# Autodesk Inventor assembly: HarmonicDrive
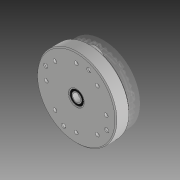
[picture p0: Inventor's stored thumbnail of the model, 180x180]
Saved by Autodesk Inventor 2020 (Build 240168000, 168)
## iProperties
Created: 2021-03-19
Part Number: HarmonicDrive
Document SubType Name: Assembly
Designer: DDeGo
Author: DDeGo
## Documents named in this file (10)
- C:\Users\DDeGo\Documents\Drew\Projects\OS-ARM\cad\HarmonicDrive75mm\HarmonicDrive.iam
- C:\Users\DDeGo\Documents\Drew\Projects\OS-ARM\cad\HarmonicDrive75mm\HD_housing.ipt
- C:\Users\DDeGo\Documents\Drew\Projects\OS-ARM\cad\HarmonicDrive75mm\HD_rotor.ipt
- C:\Users\DDeGo\Documents\Drew\Projects\OS-ARM\cad\OTS\608 bearing.ipt
- C:\Users\DDeGo\Documents\Drew\Projects\OS-ARM\cad\HarmonicDrive75mm\HD_housing2.ipt
- C:\Users\DDeGo\Documents\Drew\Projects\OS-ARM\cad\HarmonicDrive75mm\HD_Spacer.ipt
- C:\Users\DDeGo\Documents\Drew\Projects\OS-ARM\cad\HarmonicDrive75mm\HD_BearingShaft1.ipt
- C:\Users\DDeGo\Documents\Drew\Projects\OS-ARM\cad\HarmonicDrive75mm\HD_BearingShaft2.ipt
- C:\Users\DDeGo\Documents\Drew\Projects\OS-ARM\cad\HarmonicDrive75mm\HD_rotorshim.ipt
- C:\Users\DDeGo\Documents\Drew\Projects\OS-ARM\cad\OTS\688 bearing.ipt
## Components (18 placed, 9 different names)
1. HD_housing:1 — Mate:53, Mate:54, Mate:57, Mate:60
2. HD_rotor:1 — Mate:4, Mate:5, Mate:9, Mate:11, Mate:23, Mate:24, Rotation:1, Mate:45, Mate:46, Mate:49, Mate:50, Mate:61
3. HD_housing2:1 — Rotation:1, Mate:53, Mate:58, Mate:59, Mate:60
4. 608 bearing:2 — Mate:5, Mate:34, Mate:38, Mate:47
5. 608 bearing:3 — Mate:4, Mate:36, Mate:39, Mate:48
6. 608 bearing:5 — Mate:9, Mate:33, Mate:37, Mate:51
7. 608 bearing:6 — Mate:11, Mate:35, Mate:40, Mate:52
8. HD_Spacer:1 — Mate:23, Mate:24, Mate:62
9. HD_BearingShaft1:1 — Mate:35, Mate:40
10. HD_BearingShaft2:1 — Mate:33, Mate:37, Mate:41, Mate:42
11. HD_BearingShaft1:2 — Mate:36, Mate:39
12. HD_BearingShaft2:2 — Mate:34, Mate:38, Mate:43, Mate:44
13. HD_rotorshim:1 — Mate:41, Mate:49, Mate:51
14. HD_rotorshim:2 — Mate:42, Mate:50, Mate:52
15. HD_rotorshim:3 — Mate:43, Mate:45, Mate:47
16. HD_rotorshim:4 — Mate:44, Mate:46, Mate:48
17. 688 bearing:1 — Mate:54, Mate:57, Mate:61, Mate:62
18. 688 bearing:2 — Mate:58, Mate:59
## Relationships (35: Mate 34, RelateRotation 1)
- Mate:4: HD_rotor:1 ↔ 608 bearing:3
- Mate:5: HD_rotor:1 ↔ 608 bearing:2
- Mate:9: HD_rotor:1 ↔ 608 bearing:5
- Mate:11: HD_rotor:1 ↔ 608 bearing:6
- Mate:23: HD_rotor:1 ↔ HD_Spacer:1
- Mate:24: HD_rotor:1 ↔ HD_Spacer:1
- Rotation:1 [RelateRotation] (20.5 ul): HD_rotor:1 ↔ HD_housing2:1
- Mate:33: 608 bearing:5 ↔ HD_BearingShaft2:1
- Mate:34: 608 bearing:2 ↔ HD_BearingShaft2:2
- Mate:35: 608 bearing:6 ↔ HD_BearingShaft1:1
- Mate:36: 608 bearing:3 ↔ HD_BearingShaft1:2
- Mate:37: 608 bearing:5 ↔ HD_BearingShaft2:1
- Mate:38: 608 bearing:2 ↔ HD_BearingShaft2:2
- Mate:39: 608 bearing:3 ↔ HD_BearingShaft1:2
- Mate:40: 608 bearing:6 ↔ HD_BearingShaft1:1
- Mate:41: HD_BearingShaft2:1 ↔ HD_rotorshim:1
- Mate:42: HD_BearingShaft2:1 ↔ HD_rotorshim:2
- Mate:43: HD_BearingShaft2:2 ↔ HD_rotorshim:3
- Mate:44: HD_BearingShaft2:2 ↔ HD_rotorshim:4
- Mate:45: HD_rotor:1 ↔ HD_rotorshim:3
- Mate:46: HD_rotor:1 ↔ HD_rotorshim:4
- Mate:47: 608 bearing:2 ↔ HD_rotorshim:3
- Mate:48: 608 bearing:3 ↔ HD_rotorshim:4
- Mate:49: HD_rotor:1 ↔ HD_rotorshim:1
- Mate:50: HD_rotor:1 ↔ HD_rotorshim:2
- Mate:51: 608 bearing:5 ↔ HD_rotorshim:1
- Mate:52: 608 bearing:6 ↔ HD_rotorshim:2
- Mate:53 (1 mm): HD_housing:1 ↔ HD_housing2:1
- Mate:54: HD_housing:1 ↔ 688 bearing:1
- Mate:57: HD_housing:1 ↔ 688 bearing:1
- Mate:58: HD_housing2:1 ↔ 688 bearing:2
- Mate:59: HD_housing2:1 ↔ 688 bearing:2
- Mate:60: HD_housing:1 ↔ HD_housing2:1
- Mate:61: HD_rotor:1 ↔ 688 bearing:1
- Mate:62: HD_Spacer:1 ↔ 688 bearing:1
